# Autodesk Inventor assembly: Mechunam base 1.10
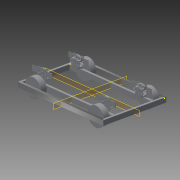
[picture p0: Inventor's stored thumbnail of the model, 180x180]
Saved by Autodesk Inventor 2015 (Build 190159000, 159)
## iProperties
Created: 2015-01-11
Part Number: Mechunam base 1.10
Document SubType Name: Weldment
Designer: chapale16
Weld Material: Welded Aluminum-6061
Author: chapale16
## Documents named in this file (11)
- \\lhssvr02\Homedirs\Robotics Club\CAD Model 2015\Mechunam base 1.10.iam
- H:\42in 2x1 boxbeam.ipt
- H:\40in 2x1 boxbeam.ipt
- H:\28in 1x2.ipt
- H:\28in 1x2_MIR1_MIR.ipt
- H:\42in 2x1 boxbeam_MIR1_MIR.ipt
- H:\Mechanum.ipt
- H:\Toughbox-mini_MIR.iam
- H:\Toughbox-mini_MIR_MIR.iam
- H:\Toughbox-mini_MIR_MIR1.iam
- H:\Toughbox-mini_MIR_MIR_MIR.iam
## Components (14 placed, 10 different names)
1. 28in 1x2:1 — Mate:1, Mate:2, Mate:24, Symmetry:1
2. 42in 2x1 boxbeam:2 — Mate:1, Mate:2, Mate:17, Mate:18, Mate:19, Mate:20, Mate:21, Symmetry:2
3. 28in 1x2_MIR1_MIR:1 — Mate:15, Mate:16, Mate:17, Mate:18, Mate:23, Symmetry:1
4. 42in 2x1 boxbeam_MIR1_MIR:1 — Mate:15, Mate:16, Symmetry:2
5. Mechanum:1 — Mate:19, Mate:21
6. Mechanum:2 — Mate:20, Mate:25
7. Mechanum:3 — Mate:22
8. Mechanum:4
9. 40in 2x1 boxbeam:1 — Mate:24, Mate:25
10. 40in 2x1 boxbeam:2 — Mate:22, Mate:23, Mate:26
11. Toughbox-mini_MIR:1 [sub-assembly] — Mate:26
12. Toughbox-mini_MIR_MIR:1 [sub-assembly]
13. Toughbox-mini_MIR_MIR1:1 [sub-assembly]
14. Toughbox-mini_MIR_MIR_MIR:1 [sub-assembly]
## Relationships (16: Mate 14, Symmetry 2)
- Mate:1: 28in 1x2:1 ↔ 42in 2x1 boxbeam:2
- Mate:2: 28in 1x2:1 ↔ 42in 2x1 boxbeam:2
- Mate:15: 28in 1x2_MIR1_MIR:1 ↔ 42in 2x1 boxbeam_MIR1_MIR:1
- Mate:16: 28in 1x2_MIR1_MIR:1 ↔ 42in 2x1 boxbeam_MIR1_MIR:1
- Mate:17: 42in 2x1 boxbeam:2 ↔ 28in 1x2_MIR1_MIR:1
- Mate:18: 42in 2x1 boxbeam:2 ↔ 28in 1x2_MIR1_MIR:1
- Mate:19 (17.145 mm): 42in 2x1 boxbeam:2 ↔ Mechanum:1
- Mate:20 (42.545 mm): 42in 2x1 boxbeam:2 ↔ Mechanum:2
- Mate:21 (42.545 mm): 42in 2x1 boxbeam:2 ↔ Mechanum:1
- Mate:22 (17.145 mm): Mechanum:3 ↔ 40in 2x1 boxbeam:2
- Mate:23: 28in 1x2_MIR1_MIR:1 ↔ 40in 2x1 boxbeam:2
- Mate:24: 28in 1x2:1 ↔ 40in 2x1 boxbeam:1
- Mate:25 (17.145 mm): Mechanum:2 ↔ 40in 2x1 boxbeam:1
- Mate:26: 40in 2x1 boxbeam:2 ↔ Toughbox-mini_MIR:1
- Symmetry:1: 28in 1x2:1 ↔ 28in 1x2_MIR1_MIR:1
- Symmetry:2: 42in 2x1 boxbeam:2 ↔ 42in 2x1 boxbeam_MIR1_MIR:1
